# Autodesk Inventor assembly: Orangatang_Kegel
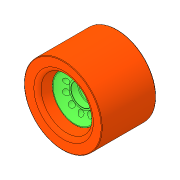
[picture p0: Inventor's stored thumbnail of the model, 180x180]
Saved by Autodesk Inventor 2017 (Build 210142000, 142)
## iProperties
Created: 2018-07-26
Part Number: Orangatang_Kegel
Document SubType Name: Assembly
Designer: Tobias
Mass: 249.775 g
Surface Area: 424.52 cm^2
Volume: 204.752 cm^3
Density: 1.21989 g/cm^3
Author: Tobias
## Documents named in this file (3)
- C:\Users\Tobias\cloudstor\CAD models\LB_project\Skate wheels\Orangatang_Kegel.iam
- C:\Users\Tobias\cloudstor\CAD models\LB_project\Skate wheels\Kegel_core.ipt
- C:\Users\Tobias\cloudstor\CAD models\LB_project\Skate wheels\Kegel_urethane.ipt
## Components (2 placed, 2 different names)
1. Kegel_core:1 — Mate:1, Flush:3, Flush:4, Mate:4, Mate:5, Mate:6
2. Kegel_urethane:1 — Mate:4, Mate:5, Mate:6
## Relationships (6: Mate 4, Flush 2)
- Mate:1: Kegel_core:1
- Flush:3: Kegel_core:1
- Flush:4: Kegel_core:1
- Mate:4: Kegel_core:1 ↔ Kegel_urethane:1
- Mate:5: Kegel_core:1 ↔ Kegel_urethane:1
- Mate:6: Kegel_core:1 ↔ Kegel_urethane:1
